# Autodesk Inventor assembly: Assembly1
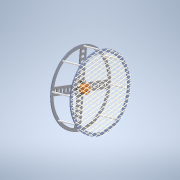
[picture p0: Inventor's stored thumbnail of the model, 180x180]
Saved by Autodesk Inventor 2021 (Build 250183000, 183)
## iProperties
Created: 2023-10-20
Part Number: Assembly1
Document SubType Name: Assembly
Designer: Lenovo
Mass: 216.424 g
Surface Area: 1443.24 cm^2
Volume: 135.689 cm^3
Density: 1.59499 g/cm^3
Author: Lenovo
## Documents named in this file (5)
- E:\0 semester 10\GP2\2DOF_Hover\CAD\Workspaces\Workspace\Assembly1.iam
- E:\0 semester 10\GP2\2DOF_Hover\CAD\Workspaces\Workspace\Part1.ipt
- E:\0 semester 10\GP2\2DOF_Hover\CAD\Workspaces\Workspace\Part18.ipt
- E:\0 semester 10\GP2\2DOF_Hover\CAD\Workspaces\Workspace\Standoff M3 M-M H 45mm.ipt
- E:\0 semester 10\GP2\2DOF_Hover\CAD\Workspaces\Workspace\guard.ipt
## Components (7 placed, 4 different names)
1. Part1:1 — Mate:25, Mate:26, Mate:27
2. Part18:1 — Mate:25, Mate:26, Mate:27, Mate:28, Mate:29, Mate:30
3. Standoff M3 M-M H 45mm:1 — Mate:33, Mate:34
4. Standoff M3 M-M H 45mm:2 — Mate:31, Mate:32
5. Standoff M3 M-M H 45mm:3 — Mate:35, Mate:36
6. Standoff M3 M-M H 45mm:4 — Mate:37, Mate:38
7. guard:1 — Mate:28, Mate:29, Mate:30, Mate:31, Mate:32, Mate:33, Mate:34, Mate:35, Mate:36, Mate:37, Mate:38
## Relationships (14: Mate 14)
- Mate:25: Part1:1 ↔ Part18:1
- Mate:26: Part1:1 ↔ Part18:1
- Mate:27: Part1:1 ↔ Part18:1
- Mate:28: Part18:1 ↔ guard:1
- Mate:29: Part18:1 ↔ guard:1
- Mate:30: Part18:1 ↔ guard:1
- Mate:31: Standoff M3 M-M H 45mm:2 ↔ guard:1
- Mate:32: Standoff M3 M-M H 45mm:2 ↔ guard:1
- Mate:33: Standoff M3 M-M H 45mm:1 ↔ guard:1
- Mate:34: Standoff M3 M-M H 45mm:1 ↔ guard:1
- Mate:35: Standoff M3 M-M H 45mm:3 ↔ guard:1
- Mate:36: Standoff M3 M-M H 45mm:3 ↔ guard:1
- Mate:37: Standoff M3 M-M H 45mm:4 ↔ guard:1
- Mate:38: Standoff M3 M-M H 45mm:4 ↔ guard:1
